# Autodesk Inventor assembly: Shoulder
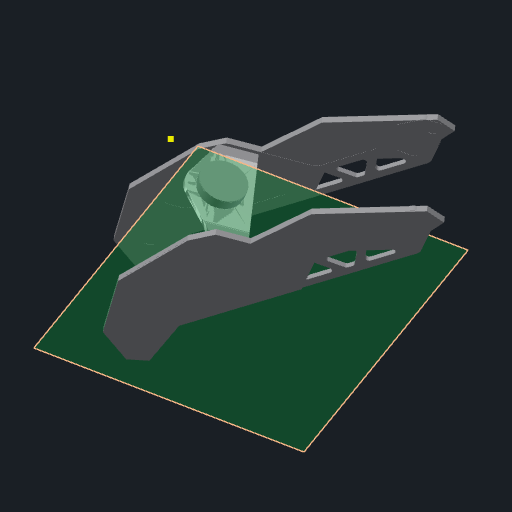
[picture p0: Inventor's stored thumbnail of the model, 512x512]
Saved by Autodesk Inventor 2025.2 (Build 292293000, 293)
## iProperties
Created: 2020-03-24
Part Number: Shoulder
Document SubType Name: Assembly
Designer: valer
Mass: 383.584 g
Surface Area: 442.479 cm^2
Volume: 56.5483 cm^3
Density: 6.7833 g/cm^3
Author: valer
## Documents named in this file (5)
- C:\Users\valer\Desktop\str1ker\cad\Shoulder.iam
- C:\Users\valer\Desktop\str1ker\cad\UpperArmBracket.ipt
- C:\Users\valer\Desktop\str1ker\cad\UpperArmBracketBase.ipt
- C:\Users\valer\Desktop\str1ker\cad\ShoulderBoundingBox.ipt
- C:\Users\valer\Desktop\str1ker\cad\ShoulderHub.ipt
## Components (5 placed, 4 different names)
1. UpperArmBracketBase:1 — Angle:2, Mate:394, Mate:395, Mate:396, Flush:1, Mate:398, Mate:399, Mate:400, Mate:401, Mate:402, Mate:403, Mate:404, Mate:405
2. ShoulderHub:1 — Mate:394, Mate:395, Mate:396, Mate:397
3. ShoulderBoundingBox:1 — Mate:397, Flush:1
4. UpperArmBracket:1 — Mate:401, Mate:402, Mate:403, Mate:404
5. UpperArmBracket:2 — Mate:399, Mate:400, Mate:405, Angle:3
## Relationships (15: Mate 12, Angle 2, Flush 1)
- Angle:2 (0 deg): UpperArmBracketBase:1
- Mate:394: UpperArmBracketBase:1 ↔ ShoulderHub:1
- Mate:395: UpperArmBracketBase:1 ↔ ShoulderHub:1
- Mate:396: UpperArmBracketBase:1 ↔ ShoulderHub:1
- Mate:397: ShoulderHub:1 ↔ ShoulderBoundingBox:1
- Flush:1: UpperArmBracketBase:1 ↔ ShoulderBoundingBox:1
- Mate:398: UpperArmBracketBase:1
- Mate:399: UpperArmBracketBase:1 ↔ UpperArmBracket:2
- Mate:400: UpperArmBracketBase:1 ↔ UpperArmBracket:2
- Mate:401: UpperArmBracketBase:1 ↔ UpperArmBracket:1
- Mate:402: UpperArmBracketBase:1 ↔ UpperArmBracket:1
- Mate:403: UpperArmBracketBase:1 ↔ UpperArmBracket:1
- Mate:404: UpperArmBracketBase:1 ↔ UpperArmBracket:1
- Mate:405: UpperArmBracketBase:1 ↔ UpperArmBracket:2
- Angle:3 (0 deg): UpperArmBracket:2
